# Autodesk Inventor assembly: plate
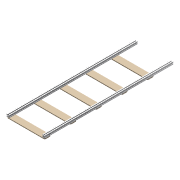
[picture p0: Inventor's stored thumbnail of the model, 180x180]
Saved by Autodesk Inventor 2017 (Build 210142000, 142)
## iProperties
Created: 2017-03-01
Part Number: plate
Document SubType Name: Assembly
Designer: sawaiz
Author: sawaiz
## Documents named in this file (5)
- C:\Users\sawaiz\oneDrive\projects\sPhenixTileTestStand\plate\plate.iam
- C:\Users\sawaiz\oneDrive\projects\sPhenixTileTestStand\plate\hfs5-2020Depth.ipt
- C:\Users\sawaiz\oneDrive\projects\sPhenixTileTestStand\plate\supportPlate.iam
- C:\Users\sawaiz\oneDrive\projects\sPhenixTileTestStand\hardware\setNut.iam
- C:\Users\sawaiz\oneDrive\projects\sPhenixTileTestStand\sPhenixTileTestStand.xlsx
## Components (9 placed, 3 different names)
1. hfs5-2020Depth:1 — Flush:1, Flush:2, Symmetry:1, Symmetry:2, Symmetry:3, Mate:1, Flush:3, Flush:4, Mate:2, Mate:3, Mate:4
2. hfs5-2020Depth:2 — Flush:1, Flush:2, Symmetry:1, Symmetry:2, Symmetry:3, Flush:5, Mate:5, Mate:6, Flush:6
3. setNut:1 [sub-assembly] — Mate:2, Mate:3, Mate:4
4. setNut:2 [sub-assembly] — Mate:5, Mate:6, Flush:6
5. supportPlate:1 [sub-assembly] — Mate:1, Flush:3, Flush:4, Flush:5
6. supportPlate:2 [sub-assembly]
7. supportPlate:3 [sub-assembly]
8. supportPlate:4 [sub-assembly]
9. supportPlate:5 [sub-assembly]
## Component patterns: (5 elements, first: supportPlate:1)
## Relationships (15: Flush 6, Mate 6, Symmetry 3)
- Flush:1: hfs5-2020Depth:1 ↔ hfs5-2020Depth:2
- Flush:2: hfs5-2020Depth:1 ↔ hfs5-2020Depth:2
- Symmetry:1: hfs5-2020Depth:1 ↔ hfs5-2020Depth:2
- Symmetry:2: hfs5-2020Depth:1 ↔ hfs5-2020Depth:2
- Symmetry:3: hfs5-2020Depth:1 ↔ hfs5-2020Depth:2
- Mate:1: hfs5-2020Depth:1 ↔ supportPlate:1
- Flush:3: hfs5-2020Depth:1 ↔ supportPlate:1
- Flush:4: hfs5-2020Depth:1 ↔ supportPlate:1
- Flush:5: hfs5-2020Depth:2 ↔ supportPlate:1
- Mate:2: hfs5-2020Depth:1 ↔ setNut:1
- Mate:3 (1 mm): hfs5-2020Depth:1 ↔ setNut:1
- Mate:4 (-40 mm): hfs5-2020Depth:1 ↔ setNut:1
- Mate:5: hfs5-2020Depth:2 ↔ setNut:2
- Mate:6 (1 mm): hfs5-2020Depth:2 ↔ setNut:2
- Flush:6 (40 mm): hfs5-2020Depth:2 ↔ setNut:2
## Named parameters: plateWidth = 300 mm, plateDepth = 1000 mm, supportPlateThickness = 6.35 mm, supportPlateWidth = 50 mm, supportPlateFillet = 10 mm, numPanels = 5, separation = 35 mm, centerVerticalRatio = 0.3
